# Autodesk Inventor assembly: Motor Assembly
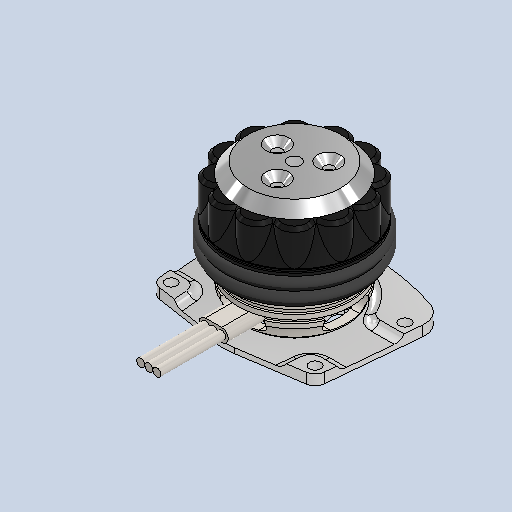
[picture p0: Inventor's stored thumbnail of the model, 512x512]
Saved by Autodesk Inventor 2023.2 (Build 272271000, 271)
## iProperties
Created: 2022-12-29
Part Number: Motor Assembly
Document SubType Name: Assembly
Designer: Nathan Cai
Mass: 129.84 g
Surface Area: 310.755 cm^2
Volume: 38.0182 cm^3
Density: 3.4152 g/cm^3
Author: Nathan Cai
## Documents named in this file (9)
- E:\Documents\Inventor\Moon Cake V0.19\Motor Assembly.iam
- E:\Documents\Inventor\Moon Cake V0.19\Motor Plate.ipt
- E:\Documents\Inventor\Moon Cake V0.19\Band - Hub.ipt
- E:\Documents\Inventor\Moon Cake V0.19\Flash_Hobby_D3536EVO v3\Flash_Hobby_D3536EVO v3.iam
- E:\Documents\Inventor\Moon Cake V0.19\Hub Cap.ipt
- E:\Documents\Inventor\Moon Cake V0.19\Band.ipt
- E:\Documents\Inventor\Moon Cake V0.19\Weapon Mold.ipt
- E:\Documents\Inventor\Moon Cake V0.19\Band - Hub - ORing.ipt
- E:\Documents\Inventor\Moon Cake V0.19\ORing 222 G40.ipt
## Components (9 placed, 8 different names)
1. Motor Plate:1 — Mate:26
2. Flash_Hobby_D3536EVO v3:2 [sub-assembly] — Mate:34, Mate:41, Mate:44, Mate:46
3. Hub Cap:1 — Mate:34, Mate:41, Mate:45
4. Band:1 — Mate:37, Mate:38
5. Band - Hub:1 — Mate:26, Mate:37, Mate:38, Mate:39, Mate:40
6. Weapon Mold:1 — Mate:39, Mate:40
7. Band - Hub - ORing:1 — Mate:42, Mate:43, Mate:44, Mate:45, Mate:46
8. ORing 222 G40:1 — Mate:43
9. ORing 222 G40:2 — Mate:42
## Relationships (15: Mate 15)
- Mate:26 (12.7 mm): Motor Plate:1 ↔ Band - Hub:1
- [Mate]: Motor Plate:1 ↔ Flash_Hobby_D3536EVO v3:2
- [Mate]: Motor Plate:1 ↔ Flash_Hobby_D3536EVO v3:2
- [Mate]: Motor Plate:1 ↔ Flash_Hobby_D3536EVO v3:2
- Mate:34: Flash_Hobby_D3536EVO v3:2 ↔ Hub Cap:1
- Mate:37: Band:1 ↔ Band - Hub:1
- Mate:38: Band:1 ↔ Band - Hub:1
- Mate:39: Band - Hub:1 ↔ Weapon Mold:1
- Mate:40: Band - Hub:1 ↔ Weapon Mold:1
- Mate:41: Flash_Hobby_D3536EVO v3:2 ↔ Hub Cap:1
- Mate:42: Band - Hub - ORing:1 ↔ ORing 222 G40:2
- Mate:43: Band - Hub - ORing:1 ↔ ORing 222 G40:1
- Mate:44: Flash_Hobby_D3536EVO v3:2 ↔ Band - Hub - ORing:1
- Mate:45: Hub Cap:1 ↔ Band - Hub - ORing:1
- Mate:46: Flash_Hobby_D3536EVO v3:2 ↔ Band - Hub - ORing:1
